# Autodesk Inventor assembly: 2AM-17-A-2200 - slider outside
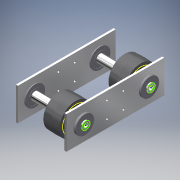
[picture p0: Inventor's stored thumbnail of the model, 180x180]
Saved by Autodesk Inventor 2017 (Build 210142000, 142)
## iProperties
Created: 2017-12-27
Part Number: 2AM-17-A-2200 - slider outside
Document SubType Name: Assembly
Designer: Micah
Author: Micah
## Documents named in this file (4)
- C:\Users\Micah\Desktop\inventor\CADathon-2017\2AM-17-A-0200 - Smokestack Elevator\2AM-17-A-2200 - slider outside.iam
- C:\Users\Micah\Desktop\inventor\CADathon-2017\2AM-17-A-0200 - Smokestack Elevator\2AM-17-A-3200 - wheels for outside slider.iam
- C:\Users\Micah\Desktop\inventor\CADathon-2017\2AM-17-A-0200 - Smokestack Elevator\2AM-17-P-2201  - slider plate.ipt
- C:\Users\Micah\Desktop\inventor\CADathon-2017\2AM-17-A-0200 - Smokestack Elevator\COTS\0_500_ID_x_1_125_OD_x_0_313_WD_Flanged_Bearing_217-2731.ipt
## Components (8 placed, 3 different names)
1. 2AM-17-P-2201  - slider plate:1 — Mate:1, Mate:2
2. 2AM-17-P-2201  - slider plate:2 — Mate:3, Mate:4
3. 0_500_ID_x_1_125_OD_x_0_313_WD_Flanged_Bearing_217-2731:1 — Mate:1, Rotational:1
4. 0_500_ID_x_1_125_OD_x_0_313_WD_Flanged_Bearing_217-2731:2 — Mate:2, Rotational:2
5. 0_500_ID_x_1_125_OD_x_0_313_WD_Flanged_Bearing_217-2731:3 — Mate:3, Insert:1
6. 0_500_ID_x_1_125_OD_x_0_313_WD_Flanged_Bearing_217-2731:4 — Mate:4, Insert:2
7. 2AM-17-A-3200 - wheels for outside slider:1 [sub-assembly] — Rotational:1, Insert:2
8. 2AM-17-A-3200 - wheels for outside slider:2 [sub-assembly] — Rotational:2, Insert:1
## Relationships (8: Mate 4, RevoluteJoint 2, Insert 2)
- Mate:1: 2AM-17-P-2201  - slider plate:1 ↔ 0_500_ID_x_1_125_OD_x_0_313_WD_Flanged_Bearing_217-2731:1
- Mate:2: 2AM-17-P-2201  - slider plate:1 ↔ 0_500_ID_x_1_125_OD_x_0_313_WD_Flanged_Bearing_217-2731:2
- Mate:3: 2AM-17-P-2201  - slider plate:2 ↔ 0_500_ID_x_1_125_OD_x_0_313_WD_Flanged_Bearing_217-2731:3
- Mate:4: 2AM-17-P-2201  - slider plate:2 ↔ 0_500_ID_x_1_125_OD_x_0_313_WD_Flanged_Bearing_217-2731:4
- Rotational:1 [RevoluteJoint] (-9.525 mm): 0_500_ID_x_1_125_OD_x_0_313_WD_Flanged_Bearing_217-2731:1 ↔ 2AM-17-A-3200 - wheels for outside slider:1
- Rotational:2 [RevoluteJoint] (-9.525 mm): 0_500_ID_x_1_125_OD_x_0_313_WD_Flanged_Bearing_217-2731:2 ↔ 2AM-17-A-3200 - wheels for outside slider:2
- Insert:1 (-9.525 mm): 0_500_ID_x_1_125_OD_x_0_313_WD_Flanged_Bearing_217-2731:3 ↔ 2AM-17-A-3200 - wheels for outside slider:2
- Insert:2 (-9.525 mm): 0_500_ID_x_1_125_OD_x_0_313_WD_Flanged_Bearing_217-2731:4 ↔ 2AM-17-A-3200 - wheels for outside slider:1
